# Autodesk Inventor assembly: blob_all
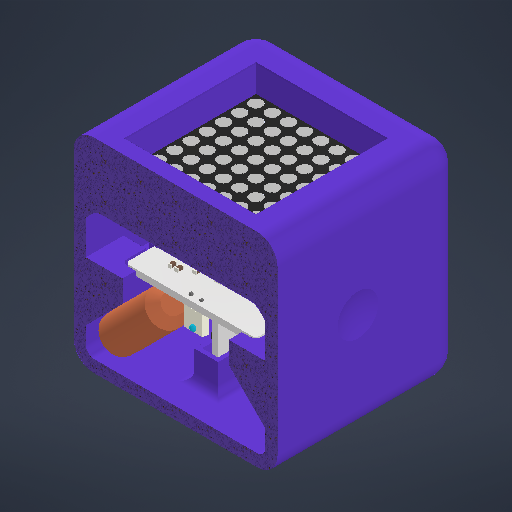
[picture p0: Inventor's stored thumbnail of the model, 512x512]
Saved by Autodesk Inventor 2025.2 (Build 292293000, 293)
## iProperties
Created: 2025-06-28
Part Number: blob_all
Document SubType Name: Assembly
Designer: micyg
Author: micyg
## Documents named in this file (6)
- D:\Projects\VirtualPets\VirtualBlob\Mechanical\blob_all.iam
- D:\Projects\VirtualPets\VirtualBlob\Mechanical\matrix\matrix.iam
- D:\Projects\VirtualPets\VirtualBlob\Mechanical\case1.ipt
- D:\Projects\VirtualPets\VirtualBlob\Mechanical\battery.ipt
- D:\Projects\VirtualPets\VirtualBlob\Mechanical\boards\mainboard_0_3_0\mainboard_0_3_0.iam
- D:\Projects\VirtualPets\VirtualBlob\Mechanical\boards\PowerBoard_0_3_0\PowerBoard_0_3_0.iam
## Components (5 placed, 5 different names)
1. case1:1 — Angle:1, Mate:18, Mate:19, Mate:20, Mate:28, Mate:29, Mate:30
2. battery:1 — Angle:1, Mate:18, Mate:19, Mate:20
3. mainboard_0_3_0:1 [sub-assembly] — Mate:22, Mate:23, Mate:24, Mate:25, Mate:26, Mate:27
4. PowerBoard_0_3_0:1 [sub-assembly] — Mate:22, Mate:23, Mate:24, Mate:30
5. matrix:2 [sub-assembly] — Mate:25, Mate:26, Mate:27, Mate:28, Mate:29
## Relationships (13: Mate 12, Angle 1)
- Angle:1 (0 deg): case1:1 ↔ battery:1
- Mate:18 (4.25 mm): case1:1 ↔ battery:1
- Mate:19: case1:1 ↔ battery:1
- Mate:20: case1:1 ↔ battery:1
- Mate:22: mainboard_0_3_0:1 ↔ PowerBoard_0_3_0:1
- Mate:23 (0.095 mm): mainboard_0_3_0:1 ↔ PowerBoard_0_3_0:1
- Mate:24 (0.1 mm): mainboard_0_3_0:1 ↔ PowerBoard_0_3_0:1
- Mate:25 (11.4 mm): mainboard_0_3_0:1 ↔ matrix:2
- Mate:26: mainboard_0_3_0:1 ↔ matrix:2
- Mate:27: mainboard_0_3_0:1 ↔ matrix:2
- Mate:28 (0.35 mm): case1:1 ↔ matrix:2
- Mate:29 (0.35 mm): case1:1 ↔ matrix:2
- Mate:30: case1:1 ↔ PowerBoard_0_3_0:1
